# Autodesk Inventor assembly: Haptic Prototyp
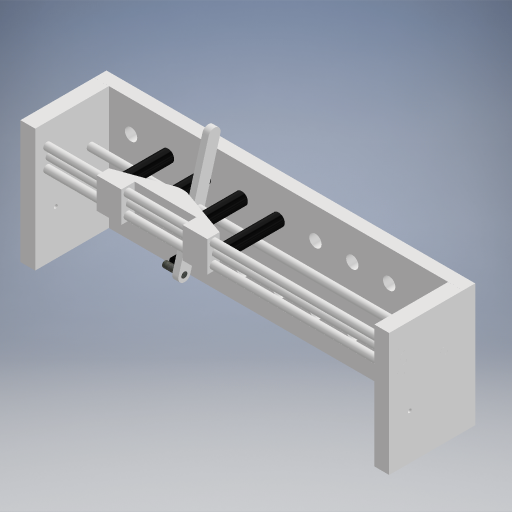
[picture p0: Inventor's stored thumbnail of the model, 512x512]
Saved by Autodesk Inventor 2024 (Build 280153000, 153)
## iProperties
Created: 2023-08-23
Part Number: Haptic Prototyp
Document SubType Name: Assembly
Designer: rapp
Author: rapp
## Documents named in this file (9)
- E:\CAD\230802 - Haptic Prototype\Haptic Prototyp.iam
- E:\CAD\230802 - Haptic Prototype\Lochplatte.ipt
- E:\CAD\230802 - Haptic Prototype\Schieber.ipt
- E:\CAD\230802 - Haptic Prototype\Hebel.ipt
- C:\Users\Vogel\Documents\Inventor\Content Center Files\R2024\de-DE\DIN ISO 8734(1)\ISO 8734 - 5 x 16 - ADIN EN.ipt
- E:\CAD\230802 - Haptic Prototype\Stift_kurz.ipt
- E:\CAD\230802 - Haptic Prototype\Stift_lang.ipt
- E:\CAD\230802 - Haptic Prototype\Seitenwand.ipt
- E:\CAD\230802 - Haptic Prototype\Führungsstange.ipt
## Components (15 placed, 8 different names)
1. Lochplatte:1 — Fluchtend:1, Passend:9, Winkel:1, Passend:10, Passend:11, Passend:12, Passend:13, Fluchtend:6, Passend:14, Fluchtend:7, Passend:15, Fluchtend:8, Fluchtend:9
2. Schieber:1 — Fluchtend:1, Winkel:1, Passend:17, Tangential:9
3. Hebel:1 — Passend:16, Tangential:8
4. DIN EN ISO 8734 5 x 16 - A:2
5. Stift_kurz:1 — Passend:9, Tangential:8
6. Stift_lang:1 — Passend:10, Tangential:9
7. Stift_lang:2 — Passend:11
8. Stift_lang:3 — Passend:12
9. Stift_lang:4 — Passend:13
10. Seitenwand:1 — Fluchtend:6, Passend:14, Fluchtend:7, Einfügen:2, Einfügen:3, Einfügen:4, Einfügen:5
11. Seitenwand:2 — Passend:15, Fluchtend:8, Fluchtend:9
12. Führungsstange:1 — Einfügen:2, Passend:17
13. Führungsstange:2 — Einfügen:3
14. Führungsstange:3 — Einfügen:4
15. Führungsstange:4 — Einfügen:5, Passend:16
## Relationships (24: Mate 10, Flush 6, Insert 4, Tangent 3, Angle 1)
- Fluchtend:1 [Flush] (12.5 mm): Lochplatte:1 ↔ Schieber:1
- [Mate]: Hebel:1 ↔ DIN EN ISO 8734 5 x 16 - A:2
- [Flush]: Hebel:1 ↔ DIN EN ISO 8734 5 x 16 - A:2
- Passend:9 [Mate]: Lochplatte:1 ↔ Stift_kurz:1
- [Tangent]: DIN EN ISO 8734 5 x 16 - A:2 ↔ Stift_kurz:1
- Winkel:1 [Angle] (0 deg): Lochplatte:1 ↔ Schieber:1
- Passend:10 [Mate]: Lochplatte:1 ↔ Stift_lang:1
- Passend:11 [Mate]: Lochplatte:1 ↔ Stift_lang:2
- Passend:12 [Mate]: Lochplatte:1 ↔ Stift_lang:3
- Passend:13 [Mate]: Lochplatte:1 ↔ Stift_lang:4
- Fluchtend:6 [Flush]: Lochplatte:1 ↔ Seitenwand:1
- Passend:14 [Mate]: Lochplatte:1 ↔ Seitenwand:1
- Fluchtend:7 [Flush]: Lochplatte:1 ↔ Seitenwand:1
- Passend:15 [Mate]: Lochplatte:1 ↔ Seitenwand:2
- Fluchtend:8 [Flush]: Lochplatte:1 ↔ Seitenwand:2
- Fluchtend:9 [Flush]: Lochplatte:1 ↔ Seitenwand:2
- Einfügen:2 [Insert]: Seitenwand:1 ↔ Führungsstange:1
- Einfügen:3 [Insert]: Seitenwand:1 ↔ Führungsstange:2
- Einfügen:4 [Insert]: Seitenwand:1 ↔ Führungsstange:3
- Einfügen:5 [Insert]: Seitenwand:1 ↔ Führungsstange:4
- Passend:16 [Mate]: Hebel:1 ↔ Führungsstange:4
- Tangential:8: Hebel:1 ↔ Stift_kurz:1
- Passend:17 [Mate]: Schieber:1 ↔ Führungsstange:1
- Tangential:9: Schieber:1 ↔ Stift_lang:1
